# Autodesk Inventor assembly: rovPrototype4
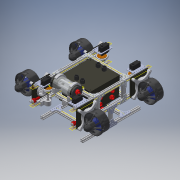
[picture p0: Inventor's stored thumbnail of the model, 180x180]
Saved by Autodesk Inventor 2018 (Build 220112000, 112)
## iProperties
Created: 2019-02-26
Part Number: rovPrototype4
Document SubType Name: Assembly
Designer: anirudh
Mass: 3427.67 g
Surface Area: 15789.2 cm^2
Volume: 2695.88 cm^3
Density: 1.27145 g/cm^3
Author: anirudh
## Documents named in this file (26)
- C:\Users\anirudh\Documents\MARS Fund\MATE Robotics\Silicon Sharks\2018-2019\Prototype4\rovPrototype4.iam
- C:\Users\anirudh\Documents\MARS Fund\MATE Robotics\Silicon Sharks\2018-2019\Prototype4\15inREV(4).ipt
- C:\Users\anirudh\Documents\MARS Fund\MATE Robotics\Silicon Sharks\2018-2019\Prototype4\LazySusanBearing(4).ipt
- C:\Users\anirudh\Documents\MARS Fund\MATE Robotics\Silicon Sharks\2018-2019\Prototype4\12inREV(4).ipt
- C:\Users\anirudh\Documents\MARS Fund\MATE Robotics\Silicon Sharks\2018-2019\Prototype4\4inREV(4).ipt
- C:\Users\anirudh\Documents\MARS Fund\Random CAD Files\REV-41-1480.ipt
- C:\Users\anirudh\Documents\MARS Fund\MATE Robotics\Silicon Sharks\2018-2019\Prototype4\ThrusterMountv2(4).ipt
- C:\Users\anirudh\Documents\MARS Fund\MATE Robotics\Silicon Sharks\2018-2019\Prototype4\BevelGearTest(4).iam
- C:\Users\anirudh\Documents\MARS Fund\Random CAD Files\REV-41-1363.ipt
- C:\Users\anirudh\Documents\MARS Fund\MATE Robotics\Silicon Sharks\2018-2019\Prototype4\Servo(4).ipt
- C:\Users\anirudh\Documents\MARS Fund\Random CAD Files\REV-41-1028.ipt
- C:\Users\anirudh\Documents\MARS Fund\MATE Robotics\Silicon Sharks\2018-2019\Prototype4\6mm-2.75inAxle(4).ipt
- C:\Users\anirudh\Documents\MARS Fund\MATE Robotics\Silicon Sharks\2018-2019\Prototype4\AxleBracket(4).ipt
- C:\Users\anirudh\Documents\MARS Fund\Random CAD Files\am-3377 6x12x4 Flanged Bearing.ipt
- C:\Users\anirudh\Documents\MARS Fund\MATE Robotics\Silicon Sharks\2018-2019\ElectronicsHousing\Prototype2\ElectricalHousing2.iam
- C:\Users\anirudh\Documents\MARS Fund\MATE Robotics\Silicon Sharks\2018-2019\Prototype4\T200-THRUSTER(4).ipt
- C:\Users\anirudh\Documents\MARS Fund\MATE Robotics\Silicon Sharks\2018-2019\CameraEnclosure\CameraEnclosure1.iam
- C:\Users\anirudh\Documents\MARS Fund\MATE Robotics\Silicon Sharks\2018-2019\Prototype4\BottomBracket.ipt
- C:\Users\anirudh\Documents\MARS Fund\MATE Robotics\Silicon Sharks\2018-2019\Prototype4\TopBracket.ipt
- C:\Users\anirudh\Documents\MARS Fund\MATE Robotics\Silicon Sharks\2018-2019\Prototype4\LED(4).ipt
- C:\Users\anirudh\Documents\MARS Fund\MATE Robotics\Silicon Sharks\2018-2019\Prototype4\IndicatorLightMount.ipt
- C:\Users\anirudh\Documents\MARS Fund\MATE Robotics\Silicon Sharks\2018-2019\Prototype4\TubeBracket.ipt
- C:\Users\anirudh\Documents\MARS Fund\MATE Robotics\Silicon Sharks\2018-2019\Prototype4\2.6inREV(4).ipt
- C:\Users\anirudh\Documents\MARS Fund\MATE Robotics\Silicon Sharks\2018-2019\Prototype4\LandingGearREV.ipt
- C:\Users\anirudh\Documents\MARS Fund\Random CAD Files\REV-41-1025.ipt
- C:\Users\anirudh\Documents\MARS Fund\MATE Robotics\Silicon Sharks\2018-2019\CameraEnclosure\CameraMount1.ipt
## Components (100 placed, 25 different names)
1. 15inREV(4):1 — Flush:1, Flush:2, Flush:3, Mate:1, Mate:2, Mate:3, Mate:5, Flush:7, Flush:8, Mate:6, Flush:9, Flush:10, Flush:44, Flush:50, Mate:94, Flush:68, Flush:74, Mate:143, Mate:144, Flush:94, Mate:146, Flush:96, Mate:168, Flush:103, Flush:104, Mate:178, Mate:180, Flush:106, Symmetry:1, Mate:191, Flush:120
2. 15inREV(4):2 — Flush:1, Flush:2, Flush:4, Flush:5, Flush:6, Mate:4, Flush:17, Flush:18, Flush:19, Flush:26, Flush:70, Flush:71, Mate:122, Flush:79, Mate:126, Flush:80, Mate:129, Flush:82, Mate:135, Flush:84, Flush:85, Flush:88
3. LazySusanBearing(4):1 — Flush:3, Mate:1, Mate:2, Flush:4, Mate:28, Mate:29, Mate:30, Mate:31, Mate:32, Mate:112
4. LazySusanBearing(4):2 — Flush:5, Flush:6, Mate:3, Mate:4, Mate:33, Mate:34, Mate:35, Mate:36, Mate:37, Mate:113
5. 12inREV(4):1 — Mate:5, Flush:7, Flush:8, Mate:12, Mate:13, Flush:43, Mate:26, Flush:48, Mate:174, Mate:177
6. 12inREV(4):2 — Mate:6, Flush:9, Flush:10, Mate:11, Mate:14, Mate:15, Flush:46, Mate:27, Flush:49, Flush:75, Mate:124
7. 15inREV(4):3 — Flush:11, Flush:12, Flush:14, Mate:8, Flush:15, Flush:16, Mate:10, Flush:17, Flush:18, Flush:22, Flush:24, Flush:61, Mate:117, Flush:63, Mate:125, Flush:77, Flush:78, Flush:81, Mate:127, Mate:131, Flush:83, Flush:90, Flush:91
8. 15inREV(4):4 — Flush:11, Flush:12, Flush:13, Mate:7, Mate:9, Mate:11, Mate:24, Mate:25, Flush:45, Flush:47, Mate:92, Flush:60, Flush:65, Flush:76, Mate:141, Mate:142, Flush:93, Mate:145, Flush:95, Mate:167, Flush:101, Flush:102, Mate:175, Symmetry:1, Mate:182, Flush:107, Flush:122
9. LazySusanBearing(4):3 — Flush:13, Mate:7, Flush:14, Mate:8, Mate:38, Mate:39, Mate:40, Mate:41, Mate:42, Mate:114
10. LazySusanBearing(4):4 — Flush:15, Flush:16, Mate:9, Mate:10, Mate:43, Mate:44, Mate:45, Mate:46, Mate:47, Mate:115
11. 4inREV(4):1 — Mate:13, Flush:22, Mate:115, Flush:64, Mate:118, Flush:66, Mate:119
12. 4inREV(4):2 — Mate:12, Flush:19, Mate:112, Flush:72, Flush:73, Mate:123
13. 4inREV(4):3 — Mate:14, Flush:24, Mate:114, Flush:59, Mate:116, Flush:62
14. 4inREV(4):4 — Mate:15, Flush:26, Mate:113, Flush:67, Mate:120, Flush:69, Mate:121
15. REV-41-1480:1 — Mate:24, Flush:43, Flush:44
16. REV-41-1480:2 — Mate:27, Flush:49, Flush:50
17. REV-41-1480:3 — Mate:25, Flush:45, Flush:46
18. REV-41-1480:4 — Mate:26, Flush:47, Flush:48
19. ThrusterMountv2(4):1 — Mate:28, Mate:29, Mate:30, Mate:31, Mate:32, Mate:50, Mate:51, Mate:148, Mate:149, Mate:150
20. ThrusterMountv2(4):2 — Mate:33, Mate:34, Mate:35, Mate:36, Mate:37, Mate:52, Mate:53, Mate:151, Mate:152, Mate:153
21. LandingGearREV:2 — Mate:186, Flush:109, Mate:187, Mate:188, Flush:110, Flush:113, Mate:190, Mate:193, Flush:114, Flush:116, Flush:119
22. ThrusterMountv2(4):3 — Mate:43, Mate:44, Mate:45, Mate:46, Mate:47, Mate:48, Mate:49, Mate:154, Mate:155, Mate:156
23. ThrusterMountv2(4):4 — Mate:38, Mate:39, Mate:40, Mate:41, Mate:42, Mate:54, Mate:55, Mate:157, Mate:158, Mate:159
24. BevelGearTest(4):1 [sub-assembly] — Mate:48, Mate:49, Mate:56, Mate:58, Mate:65, Mate:81
25. BevelGearTest(4):2 [sub-assembly] — Mate:50, Mate:51, Mate:57, Mate:59, Mate:67, Mate:83
26. BevelGearTest(4):3 [sub-assembly] — Mate:52, Mate:53, Mate:62, Mate:63, Mate:87, Mate:134
27. BevelGearTest(4):4 [sub-assembly] — Mate:54, Mate:55, Mate:60, Mate:61, Mate:69, Mate:85
28. REV-41-1363:1 — Mate:56, Mate:58, Mate:64, Mate:80
29. REV-41-1363:2 — Mate:57, Mate:59, Mate:66, Mate:82
30. REV-41-1363:3 — Mate:62, Mate:63, Mate:86, Mate:133
31. REV-41-1363:4 — Mate:60, Mate:61, Mate:68, Mate:84
32. Servo(4):1 — Mate:64, Mate:65, Mate:128
33. Servo(4):2 — Mate:66, Mate:67, Mate:130
34. Servo(4):3 — Mate:68, Mate:69, Mate:132
35. REV-41-1028:1 — Flush:81, Mate:127, Mate:128
36. REV-41-1028:2 — Mate:129, Flush:82, Mate:130
37. REV-41-1028:3 — Mate:131, Flush:83, Mate:132
38. REV-41-1028:4 — Mate:135, Flush:84, Mate:136
39. 6mm-2.75inAxle(4):1 — Mate:80, Mate:81, Mate:97, Mate:99
40. 6mm-2.75inAxle(4):2 — Mate:82, Mate:83, Mate:101, Mate:103
41. 6mm-2.75inAxle(4):3 — Mate:84, Mate:85, Mate:105, Mate:107
42. 6mm-2.75inAxle(4):4 — Mate:86, Mate:87, Mate:109, Mate:111
43. AxleBracket(4):1 — Mate:96, Mate:98, Mate:141, Mate:142, Flush:93
44. AxleBracket(4):2 — Mate:100, Mate:102, Mate:143, Mate:144, Flush:94
45. AxleBracket(4):3 — Mate:92, Mate:104, Mate:106, Mate:145, Flush:95
46. AxleBracket(4):4 — Mate:94, Mate:108, Mate:110, Mate:146, Flush:96
47. am-3377 6x12x4 Flanged Bearing:1 — Mate:96, Mate:97
48. am-3377 6x12x4 Flanged Bearing:2 — Mate:98, Mate:99
49. am-3377 6x12x4 Flanged Bearing:3 — Mate:100, Mate:101
50. am-3377 6x12x4 Flanged Bearing:4 — Mate:102, Mate:103
51. am-3377 6x12x4 Flanged Bearing:5 — Mate:106, Mate:107
52. am-3377 6x12x4 Flanged Bearing:6 — Mate:104, Mate:105
53. am-3377 6x12x4 Flanged Bearing:7 — Mate:110, Mate:111
54. am-3377 6x12x4 Flanged Bearing:8 — Mate:108, Mate:109
55. REV-41-1480:5 — Flush:59, Flush:60, Mate:116
56. REV-41-1480:6 — Flush:63, Flush:64, Mate:118
57. REV-41-1480:7 — Flush:61, Flush:62, Mate:117
58. REV-41-1480:8 — Flush:65, Flush:66, Mate:119
59. REV-41-1480:9 — Flush:71, Mate:122, Flush:72
60. REV-41-1480:10 — Flush:73, Flush:74, Mate:123
61. REV-41-1480:11 — Flush:67, Mate:120, Flush:68
62. REV-41-1480:12 — Flush:69, Flush:70, Mate:121
63. ElectricalHousing2:1 [sub-assembly] — Flush:75, Flush:76, Mate:124, Mate:173, Mate:176
64. 12inREV(4):3 — Flush:79, Mate:126, Flush:80, Flush:87, Mate:138, Flush:92, Mate:140
65. 12inREV(4):4 — Mate:125, Flush:77, Flush:78, Flush:86, Mate:137, Flush:89, Mate:139, Mate:160, Mate:161, Mate:162, Mate:163, Mate:165, Flush:98, Mate:166, Flush:100
66. Servo(4):4 — Mate:133, Mate:134, Mate:136
67. REV-41-1480:13 — Flush:89, Flush:90, Mate:139
68. REV-41-1480:14 — Flush:91, Flush:92, Mate:140
69. REV-41-1480:15 — Flush:85, Flush:86, Mate:137
70. REV-41-1480:16 — Flush:87, Flush:88, Mate:138
71. T200-THRUSTER(4):1 — Mate:148, Mate:149, Mate:150
72. T200-THRUSTER(4):2 — Mate:151, Mate:152, Mate:153
73. T200-THRUSTER(4):3 — Mate:154, Mate:155, Mate:156
74. T200-THRUSTER(4):4 — Mate:157, Mate:158, Mate:159
75. CameraEnclosure1:1 [sub-assembly] — Mate:164, Mate:198, Mate:199
76. BottomBracket:1 — Mate:160, Mate:163
77. BottomBracket:2 — Mate:161, Mate:162, Mate:164
78. TopBracket:1 — Mate:165, Flush:98
79. TopBracket:2 — Mate:166, Flush:100
80. LED(4):1 — Mate:169, Mate:170
81. LED(4):2 — Mate:171, Mate:172
82. IndicatorLightMount:1 — Mate:167, Flush:101, Flush:102, Mate:169, Mate:170
83. IndicatorLightMount:2 — Mate:168, Flush:103, Flush:104, Mate:171, Mate:172
84. CameraEnclosure1:2 [sub-assembly] — Flush:105, Mate:179
85. TubeBracket:1 — Mate:173, Mate:174, Mate:175, Flush:105, Mate:179
86. TubeBracket:2 — Mate:176, Mate:177, Mate:178
87. 2.6inREV(4):1 — Mate:180, Flush:106, Mate:181, Mate:186, Flush:109, Mate:187, Flush:118, Flush:121
88. 2.6inREV(4):2 — Mate:182, Mate:183, Flush:107, Mate:184, Mate:185, Flush:108, Mate:197, Flush:123, Flush:128
89. LandingGearREV:1 — Mate:184, Mate:185, Flush:108, Mate:189, Flush:111, Flush:112, Mate:194, Mate:195, Mate:196, Flush:125, Flush:127, Flush:129
90. 12inREV(4):5 — Mate:188, Flush:110, Flush:113, Mate:192, Flush:117, Flush:126
91. 12inREV(4):6 — Mate:189, Flush:111, Flush:112, Flush:115, Flush:124
92. REV-41-1025:1 — Mate:190, Flush:118, Flush:119
93. REV-41-1025:2 — Mate:191, Flush:120, Flush:121
94. REV-41-1025:3 — Mate:193, Flush:114, Flush:115
95. REV-41-1025:4 — Mate:192, Flush:116, Flush:117
96. REV-41-1025:5 — Mate:197, Flush:122, Flush:123
97. REV-41-1025:6 — Mate:195, Flush:126, Flush:127
98. REV-41-1025:7 — Mate:196, Flush:128, Flush:129
99. REV-41-1025:8 — Mate:194, Flush:124, Flush:125
100. CameraMount1:1 — Mate:198, Mate:199
## Relationships (274: Mate 174, Flush 99, Symmetry 1)
- Flush:1: 15inREV(4):1 ↔ 15inREV(4):2
- Flush:2: 15inREV(4):1 ↔ 15inREV(4):2
- Flush:3: 15inREV(4):1 ↔ LazySusanBearing(4):1
- Mate:1: 15inREV(4):1 ↔ LazySusanBearing(4):1
- Mate:2: 15inREV(4):1 ↔ LazySusanBearing(4):1
- Flush:4: 15inREV(4):2 ↔ LazySusanBearing(4):1
- Flush:5: 15inREV(4):2 ↔ LazySusanBearing(4):2
- Flush:6: 15inREV(4):2 ↔ LazySusanBearing(4):2
- Mate:3: 15inREV(4):1 ↔ LazySusanBearing(4):2
- Mate:4: 15inREV(4):2 ↔ LazySusanBearing(4):2
- Mate:5: 15inREV(4):1 ↔ 12inREV(4):1
- Flush:7: 15inREV(4):1 ↔ 12inREV(4):1
- Flush:8 (97.282 mm): 15inREV(4):1 ↔ 12inREV(4):1
- Mate:6: 15inREV(4):1 ↔ 12inREV(4):2
- Flush:9: 15inREV(4):1 ↔ 12inREV(4):2
- Flush:10 (97.282 mm): 15inREV(4):1 ↔ 12inREV(4):2
- Flush:11: 15inREV(4):3 ↔ 15inREV(4):4
- Flush:12: 15inREV(4):3 ↔ 15inREV(4):4
- Flush:13: 15inREV(4):4 ↔ LazySusanBearing(4):3
- Mate:7: 15inREV(4):4 ↔ LazySusanBearing(4):3
- Flush:14: 15inREV(4):3 ↔ LazySusanBearing(4):3
- Mate:8: 15inREV(4):3 ↔ LazySusanBearing(4):3
- Flush:15: 15inREV(4):3 ↔ LazySusanBearing(4):4
- Flush:16: 15inREV(4):3 ↔ LazySusanBearing(4):4
- Mate:9: 15inREV(4):4 ↔ LazySusanBearing(4):4
- Mate:10: 15inREV(4):3 ↔ LazySusanBearing(4):4
- Flush:17: 15inREV(4):2 ↔ 15inREV(4):3
- Flush:18: 15inREV(4):2 ↔ 15inREV(4):3
- Mate:11: 12inREV(4):2 ↔ 15inREV(4):4
- Mate:12: 12inREV(4):1 ↔ 4inREV(4):2
- Flush:19: 15inREV(4):2 ↔ 4inREV(4):2
- Mate:13: 12inREV(4):1 ↔ 4inREV(4):1
- Flush:22: 15inREV(4):3 ↔ 4inREV(4):1
- Mate:14: 12inREV(4):2 ↔ 4inREV(4):3
- Flush:24: 15inREV(4):3 ↔ 4inREV(4):3
- Mate:15: 12inREV(4):2 ↔ 4inREV(4):4
- Flush:26: 15inREV(4):2 ↔ 4inREV(4):4
- Mate:24: 15inREV(4):4 ↔ REV-41-1480:1
- Flush:43: 12inREV(4):1 ↔ REV-41-1480:1
- Flush:44: 15inREV(4):1 ↔ REV-41-1480:1
- Mate:25: 15inREV(4):4 ↔ REV-41-1480:3
- Flush:45: 15inREV(4):4 ↔ REV-41-1480:3
- Flush:46: 12inREV(4):2 ↔ REV-41-1480:3
- Mate:26: 12inREV(4):1 ↔ REV-41-1480:4
- Flush:47: 15inREV(4):4 ↔ REV-41-1480:4
- Flush:48: 12inREV(4):1 ↔ REV-41-1480:4
- Mate:27: 12inREV(4):2 ↔ REV-41-1480:2
- Flush:49: 12inREV(4):2 ↔ REV-41-1480:2
- Flush:50: 15inREV(4):1 ↔ REV-41-1480:2
- Mate:28: LazySusanBearing(4):1 ↔ ThrusterMountv2(4):1
- Mate:29: LazySusanBearing(4):1 ↔ ThrusterMountv2(4):1
- Mate:30: LazySusanBearing(4):1 ↔ ThrusterMountv2(4):1
- Mate:31: LazySusanBearing(4):1 ↔ ThrusterMountv2(4):1
- Mate:32: LazySusanBearing(4):1 ↔ ThrusterMountv2(4):1
- Mate:33: LazySusanBearing(4):2 ↔ ThrusterMountv2(4):2
- Mate:34: LazySusanBearing(4):2 ↔ ThrusterMountv2(4):2
- Mate:35: LazySusanBearing(4):2 ↔ ThrusterMountv2(4):2
- Mate:36: LazySusanBearing(4):2 ↔ ThrusterMountv2(4):2
- Mate:37: LazySusanBearing(4):2 ↔ ThrusterMountv2(4):2
- Mate:38: LazySusanBearing(4):3 ↔ ThrusterMountv2(4):4
- Mate:39: LazySusanBearing(4):3 ↔ ThrusterMountv2(4):4
- Mate:40: LazySusanBearing(4):3 ↔ ThrusterMountv2(4):4
- Mate:41: LazySusanBearing(4):3 ↔ ThrusterMountv2(4):4
- Mate:42: LazySusanBearing(4):3 ↔ ThrusterMountv2(4):4
- Mate:43: LazySusanBearing(4):4 ↔ ThrusterMountv2(4):3
- Mate:44: LazySusanBearing(4):4 ↔ ThrusterMountv2(4):3
- Mate:45: LazySusanBearing(4):4 ↔ ThrusterMountv2(4):3
- Mate:46: LazySusanBearing(4):4 ↔ ThrusterMountv2(4):3
- Mate:47: LazySusanBearing(4):4 ↔ ThrusterMountv2(4):3
- Mate:48: ThrusterMountv2(4):3 ↔ BevelGearTest(4):1
- Mate:49: ThrusterMountv2(4):3 ↔ BevelGearTest(4):1
- Mate:50: ThrusterMountv2(4):1 ↔ BevelGearTest(4):2
- Mate:51: ThrusterMountv2(4):1 ↔ BevelGearTest(4):2
- Mate:52: ThrusterMountv2(4):2 ↔ BevelGearTest(4):3
- Mate:53: ThrusterMountv2(4):2 ↔ BevelGearTest(4):3
- Mate:54: ThrusterMountv2(4):4 ↔ BevelGearTest(4):4
- Mate:55: ThrusterMountv2(4):4 ↔ BevelGearTest(4):4
- Mate:56: BevelGearTest(4):1 ↔ REV-41-1363:1
- Mate:57: BevelGearTest(4):2 ↔ REV-41-1363:2
- Mate:58: BevelGearTest(4):1 ↔ REV-41-1363:1
- Mate:59: BevelGearTest(4):2 ↔ REV-41-1363:2
- Mate:60: BevelGearTest(4):4 ↔ REV-41-1363:4
- Mate:61: BevelGearTest(4):4 ↔ REV-41-1363:4
- Mate:62: BevelGearTest(4):3 ↔ REV-41-1363:3
- Mate:63: BevelGearTest(4):3 ↔ REV-41-1363:3
- Mate:64: REV-41-1363:1 ↔ Servo(4):1
- Mate:65: BevelGearTest(4):1 ↔ Servo(4):1
- Mate:66: REV-41-1363:2 ↔ Servo(4):2
- Mate:67: BevelGearTest(4):2 ↔ Servo(4):2
- Mate:68: REV-41-1363:4 ↔ Servo(4):3
- Mate:69: BevelGearTest(4):4 ↔ Servo(4):3
- Mate:80 (5.08 mm): REV-41-1363:1 ↔ 6mm-2.75inAxle(4):1
- Mate:81: BevelGearTest(4):1 ↔ 6mm-2.75inAxle(4):1
- Mate:82 (5.08 mm): REV-41-1363:2 ↔ 6mm-2.75inAxle(4):2
- Mate:83: BevelGearTest(4):2 ↔ 6mm-2.75inAxle(4):2
- Mate:84 (5.08 mm): REV-41-1363:4 ↔ 6mm-2.75inAxle(4):3
- Mate:85: BevelGearTest(4):4 ↔ 6mm-2.75inAxle(4):3
- Mate:86 (5.08 mm): REV-41-1363:3 ↔ 6mm-2.75inAxle(4):4
- Mate:87: BevelGearTest(4):3 ↔ 6mm-2.75inAxle(4):4
- Mate:92: 15inREV(4):4 ↔ AxleBracket(4):3
- Mate:94: 15inREV(4):1 ↔ AxleBracket(4):4
- Mate:96: AxleBracket(4):1 ↔ am-3377 6x12x4 Flanged Bearing:1
- Mate:97: 6mm-2.75inAxle(4):1 ↔ am-3377 6x12x4 Flanged Bearing:1
- Mate:98: AxleBracket(4):1 ↔ am-3377 6x12x4 Flanged Bearing:2
- Mate:99: 6mm-2.75inAxle(4):1 ↔ am-3377 6x12x4 Flanged Bearing:2
- Mate:100: AxleBracket(4):2 ↔ am-3377 6x12x4 Flanged Bearing:3
- Mate:101: 6mm-2.75inAxle(4):2 ↔ am-3377 6x12x4 Flanged Bearing:3
- Mate:102: AxleBracket(4):2 ↔ am-3377 6x12x4 Flanged Bearing:4
- Mate:103: 6mm-2.75inAxle(4):2 ↔ am-3377 6x12x4 Flanged Bearing:4
- Mate:104: AxleBracket(4):3 ↔ am-3377 6x12x4 Flanged Bearing:6
- Mate:105: 6mm-2.75inAxle(4):3 ↔ am-3377 6x12x4 Flanged Bearing:6
- Mate:106: AxleBracket(4):3 ↔ am-3377 6x12x4 Flanged Bearing:5
- Mate:107: 6mm-2.75inAxle(4):3 ↔ am-3377 6x12x4 Flanged Bearing:5
- Mate:108: AxleBracket(4):4 ↔ am-3377 6x12x4 Flanged Bearing:8
- Mate:109: 6mm-2.75inAxle(4):4 ↔ am-3377 6x12x4 Flanged Bearing:8
- Mate:110: AxleBracket(4):4 ↔ am-3377 6x12x4 Flanged Bearing:7
- Mate:111: 6mm-2.75inAxle(4):4 ↔ am-3377 6x12x4 Flanged Bearing:7
- Mate:112 (19.05 mm): LazySusanBearing(4):1 ↔ 4inREV(4):2
- Mate:113 (19.05 mm): LazySusanBearing(4):2 ↔ 4inREV(4):4
- Mate:114 (19.05 mm): LazySusanBearing(4):3 ↔ 4inREV(4):3
- Mate:115 (19.05 mm): LazySusanBearing(4):4 ↔ 4inREV(4):1
- Flush:59: 4inREV(4):3 ↔ REV-41-1480:5
- Flush:60: 15inREV(4):4 ↔ REV-41-1480:5
- Mate:116: 4inREV(4):3 ↔ REV-41-1480:5
- Flush:61: 15inREV(4):3 ↔ REV-41-1480:7
- Flush:62: 4inREV(4):3 ↔ REV-41-1480:7
- Mate:117: 15inREV(4):3 ↔ REV-41-1480:7
- Flush:63: 15inREV(4):3 ↔ REV-41-1480:6
- Flush:64: 4inREV(4):1 ↔ REV-41-1480:6
- Mate:118: 4inREV(4):1 ↔ REV-41-1480:6
- Flush:65: 15inREV(4):4 ↔ REV-41-1480:8
- Flush:66: 4inREV(4):1 ↔ REV-41-1480:8
- Mate:119: 4inREV(4):1 ↔ REV-41-1480:8
- Flush:67: 4inREV(4):4 ↔ REV-41-1480:11
- Mate:120: 4inREV(4):4 ↔ REV-41-1480:11
- Flush:68: 15inREV(4):1 ↔ REV-41-1480:11
- Flush:69: 4inREV(4):4 ↔ REV-41-1480:12
- Flush:70: 15inREV(4):2 ↔ REV-41-1480:12
- Mate:121: 4inREV(4):4 ↔ REV-41-1480:12
- Flush:71: 15inREV(4):2 ↔ REV-41-1480:9
- Mate:122: 15inREV(4):2 ↔ REV-41-1480:9
- Flush:72: 4inREV(4):2 ↔ REV-41-1480:9
- Flush:73: 4inREV(4):2 ↔ REV-41-1480:10
- Flush:74: 15inREV(4):1 ↔ REV-41-1480:10
- Mate:123: 4inREV(4):2 ↔ REV-41-1480:10
- Flush:75 (0.4318 mm): 12inREV(4):2 ↔ ElectricalHousing2:1
- Flush:76 (38.0238 mm): 15inREV(4):4 ↔ ElectricalHousing2:1
- Mate:124: 12inREV(4):2 ↔ ElectricalHousing2:1
- Mate:125: 15inREV(4):3 ↔ 12inREV(4):4
- Flush:77: 15inREV(4):3 ↔ 12inREV(4):4
- Flush:78 (93.98 mm): 15inREV(4):3 ↔ 12inREV(4):4
- Flush:79: 15inREV(4):2 ↔ 12inREV(4):3
- Mate:126: 15inREV(4):2 ↔ 12inREV(4):3
- Flush:80 (93.98 mm): 15inREV(4):2 ↔ 12inREV(4):3
- Flush:81: 15inREV(4):3 ↔ REV-41-1028:1
- Mate:127: 15inREV(4):3 ↔ REV-41-1028:1
- Mate:128 (1.016 mm): Servo(4):1 ↔ REV-41-1028:1
- Mate:129: 15inREV(4):2 ↔ REV-41-1028:2
- Flush:82: 15inREV(4):2 ↔ REV-41-1028:2
- Mate:130 (1.016 mm): Servo(4):2 ↔ REV-41-1028:2
- Mate:131: 15inREV(4):3 ↔ REV-41-1028:3
- Flush:83: 15inREV(4):3 ↔ REV-41-1028:3
- Mate:132 (1.016 mm): Servo(4):3 ↔ REV-41-1028:3
- Mate:133: REV-41-1363:3 ↔ Servo(4):4
- Mate:134: BevelGearTest(4):3 ↔ Servo(4):4
- Mate:135: 15inREV(4):2 ↔ REV-41-1028:4
- Flush:84: 15inREV(4):2 ↔ REV-41-1028:4
- Mate:136 (1.016 mm): REV-41-1028:4 ↔ Servo(4):4
- Flush:85: 15inREV(4):2 ↔ REV-41-1480:15
- Flush:86: 12inREV(4):4 ↔ REV-41-1480:15
- Mate:137: 12inREV(4):4 ↔ REV-41-1480:15
- Flush:87: 12inREV(4):3 ↔ REV-41-1480:16
- Flush:88: 15inREV(4):2 ↔ REV-41-1480:16
- Mate:138: 12inREV(4):3 ↔ REV-41-1480:16
- Flush:89: 12inREV(4):4 ↔ REV-41-1480:13
- Flush:90: 15inREV(4):3 ↔ REV-41-1480:13
- Mate:139: 12inREV(4):4 ↔ REV-41-1480:13
- Flush:91: 15inREV(4):3 ↔ REV-41-1480:14
- Flush:92: 12inREV(4):3 ↔ REV-41-1480:14
- Mate:140: 12inREV(4):3 ↔ REV-41-1480:14
- Mate:141: 15inREV(4):4 ↔ AxleBracket(4):1
- Mate:142: 15inREV(4):4 ↔ AxleBracket(4):1
- Flush:93 (19.9136 mm): 15inREV(4):4 ↔ AxleBracket(4):1
- Mate:143: 15inREV(4):1 ↔ AxleBracket(4):2
- Mate:144: 15inREV(4):1 ↔ AxleBracket(4):2
- Flush:94 (19.9136 mm): 15inREV(4):1 ↔ AxleBracket(4):2
- Mate:145: 15inREV(4):4 ↔ AxleBracket(4):3
- Flush:95 (19.9136 mm): 15inREV(4):4 ↔ AxleBracket(4):3
- Mate:146: 15inREV(4):1 ↔ AxleBracket(4):4
- Flush:96 (19.9136 mm): 15inREV(4):1 ↔ AxleBracket(4):4
- Mate:148: ThrusterMountv2(4):1 ↔ T200-THRUSTER(4):1
- Mate:149: ThrusterMountv2(4):1 ↔ T200-THRUSTER(4):1
- Mate:150: ThrusterMountv2(4):1 ↔ T200-THRUSTER(4):1
- Mate:151: ThrusterMountv2(4):2 ↔ T200-THRUSTER(4):2
- Mate:152: ThrusterMountv2(4):2 ↔ T200-THRUSTER(4):2
- Mate:153: ThrusterMountv2(4):2 ↔ T200-THRUSTER(4):2
- Mate:154: ThrusterMountv2(4):3 ↔ T200-THRUSTER(4):3
- Mate:155: ThrusterMountv2(4):3 ↔ T200-THRUSTER(4):3
- Mate:156: ThrusterMountv2(4):3 ↔ T200-THRUSTER(4):3
- Mate:157: ThrusterMountv2(4):4 ↔ T200-THRUSTER(4):4
- Mate:158: ThrusterMountv2(4):4 ↔ T200-THRUSTER(4):4
- Mate:159: ThrusterMountv2(4):4 ↔ T200-THRUSTER(4):4
- Mate:160: 12inREV(4):4 ↔ BottomBracket:1
- Mate:161: 12inREV(4):4 ↔ BottomBracket:2
- Mate:162: 12inREV(4):4 ↔ BottomBracket:2
- Mate:163: 12inREV(4):4 ↔ BottomBracket:1
- Mate:164: CameraEnclosure1:1 ↔ BottomBracket:2
- Mate:165: 12inREV(4):4 ↔ TopBracket:1
- Flush:98: 12inREV(4):4 ↔ TopBracket:1
- Mate:166: 12inREV(4):4 ↔ TopBracket:2
- Flush:100: 12inREV(4):4 ↔ TopBracket:2
- Mate:167: 15inREV(4):4 ↔ IndicatorLightMount:1
- Flush:101: 15inREV(4):4 ↔ IndicatorLightMount:1
- Flush:102: 15inREV(4):4 ↔ IndicatorLightMount:1
- Mate:168: 15inREV(4):1 ↔ IndicatorLightMount:2
- Flush:103: 15inREV(4):1 ↔ IndicatorLightMount:2
- Flush:104: 15inREV(4):1 ↔ IndicatorLightMount:2
- Mate:169: LED(4):1 ↔ IndicatorLightMount:1
- Mate:170: LED(4):1 ↔ IndicatorLightMount:1
- Mate:171: LED(4):2 ↔ IndicatorLightMount:2
- Mate:172: LED(4):2 ↔ IndicatorLightMount:2
- Mate:173: ElectricalHousing2:1 ↔ TubeBracket:1
- Mate:174: 12inREV(4):1 ↔ TubeBracket:1
- Mate:175 (45.974 mm): 15inREV(4):4 ↔ TubeBracket:1
- Mate:176: ElectricalHousing2:1 ↔ TubeBracket:2
- Mate:177: 12inREV(4):1 ↔ TubeBracket:2
- Mate:178 (45.974 mm): 15inREV(4):1 ↔ TubeBracket:2
- Flush:105 (-6 mm): CameraEnclosure1:2 ↔ TubeBracket:1
- Mate:179: CameraEnclosure1:2 ↔ TubeBracket:1
- Mate:180: 15inREV(4):1 ↔ 2.6inREV(4):1
- Flush:106: 15inREV(4):1 ↔ 2.6inREV(4):1
- Symmetry:1: 15inREV(4):1 ↔ 15inREV(4):4
- Mate:181: 2.6inREV(4):1
- Mate:182: 15inREV(4):4 ↔ 2.6inREV(4):2
- Mate:183: 2.6inREV(4):2
- Flush:107: 15inREV(4):4 ↔ 2.6inREV(4):2
- Mate:184: 2.6inREV(4):2 ↔ LandingGearREV:1
- Mate:185: 2.6inREV(4):2 ↔ LandingGearREV:1
- Flush:108: 2.6inREV(4):2 ↔ LandingGearREV:1
- Mate:186: LandingGearREV:2 ↔ 2.6inREV(4):1
- Flush:109: LandingGearREV:2 ↔ 2.6inREV(4):1
- Mate:187: LandingGearREV:2 ↔ 2.6inREV(4):1
- Mate:188: LandingGearREV:2 ↔ 12inREV(4):5
- Flush:110: LandingGearREV:2 ↔ 12inREV(4):5
- Mate:189: LandingGearREV:1 ↔ 12inREV(4):6
- Flush:111: LandingGearREV:1 ↔ 12inREV(4):6
- Flush:112: LandingGearREV:1 ↔ 12inREV(4):6
- Flush:113: LandingGearREV:2 ↔ 12inREV(4):5
- Mate:190: LandingGearREV:2 ↔ REV-41-1025:1
- Mate:191: 15inREV(4):1 ↔ REV-41-1025:2
- Mate:192: 12inREV(4):5 ↔ REV-41-1025:4
- Mate:193: LandingGearREV:2 ↔ REV-41-1025:3
- Flush:114: LandingGearREV:2 ↔ REV-41-1025:3
- Flush:115: 12inREV(4):6 ↔ REV-41-1025:3
- Flush:116: LandingGearREV:2 ↔ REV-41-1025:4
- Flush:117: 12inREV(4):5 ↔ REV-41-1025:4
- Flush:118: 2.6inREV(4):1 ↔ REV-41-1025:1
- Flush:119: LandingGearREV:2 ↔ REV-41-1025:1
- Flush:120: 15inREV(4):1 ↔ REV-41-1025:2
- Flush:121: 2.6inREV(4):1 ↔ REV-41-1025:2
- Mate:194: LandingGearREV:1 ↔ REV-41-1025:8
- Mate:195: LandingGearREV:1 ↔ REV-41-1025:6
- Mate:196: LandingGearREV:1 ↔ REV-41-1025:7
- Mate:197: 2.6inREV(4):2 ↔ REV-41-1025:5
- Flush:122: 15inREV(4):4 ↔ REV-41-1025:5
- Flush:123: 2.6inREV(4):2 ↔ REV-41-1025:5
- Flush:124: 12inREV(4):6 ↔ REV-41-1025:8
- Flush:125: LandingGearREV:1 ↔ REV-41-1025:8
- Flush:126: 12inREV(4):5 ↔ REV-41-1025:6
- Flush:127: LandingGearREV:1 ↔ REV-41-1025:6
- Flush:128: 2.6inREV(4):2 ↔ REV-41-1025:7
- Flush:129: LandingGearREV:1 ↔ REV-41-1025:7
- Mate:198: CameraEnclosure1:1 ↔ CameraMount1:1
- Mate:199: CameraEnclosure1:1 ↔ CameraMount1:1
